# Autodesk Inventor assembly: LCDassembly
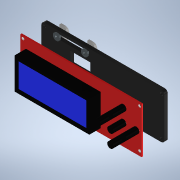
[picture p0: Inventor's stored thumbnail of the model, 180x180]
Saved by Autodesk Inventor 2020.2 (Build 242310000, 310)
## iProperties
Created: 2020-08-24
Part Number: LCDassembly
Document SubType Name: Assembly
Designer: JK
Author: JK
## Documents named in this file (5)
- C:\Users\JK\Documents\Inventor\Anet Upgrade\LCDassembly.iam
- C:\Users\JK\Documents\Inventor\Anet Upgrade\LCDmount.ipt
- C:\Users\JK\Documents\Inventor\Anet Upgrade\LCDScreen.ipt
- C:\Users\JK\Documents\Inventor\Anet Upgrade\M5x12BoltFlatHead.ipt
- C:\Users\JK\Documents\Inventor\Anet Upgrade\T_Slot_Nut_Dropin_3030m5ipt.ipt
## Components (6 placed, 4 different names)
1. LCDmount:1 — Mate:1, Mate:2, Mate:5, Mate:6, Mate:7, Mate:8
2. LCDScreen:1 — Mate:1, Mate:2
3. M5x12BoltFlatHead:1 — Flush:1, Mate:4
4. M5x12BoltFlatHead:2 — Flush:1, Mate:3
5. T_Slot_Nut_Dropin_3030m5ipt:1 — Mate:3, Flush:2, Mate:8, Flush:3
6. T_Slot_Nut_Dropin_3030m5ipt:2 — Mate:4, Flush:2, Mate:5, Mate:6, Mate:7, Flush:3
## Relationships (11: Mate 8, Flush 3)
- Mate:1: LCDmount:1 ↔ LCDScreen:1
- Mate:2: LCDmount:1 ↔ LCDScreen:1
- Flush:1: M5x12BoltFlatHead:1 ↔ M5x12BoltFlatHead:2
- Mate:3: M5x12BoltFlatHead:2 ↔ T_Slot_Nut_Dropin_3030m5ipt:1
- Mate:4: M5x12BoltFlatHead:1 ↔ T_Slot_Nut_Dropin_3030m5ipt:2
- Flush:2: T_Slot_Nut_Dropin_3030m5ipt:1 ↔ T_Slot_Nut_Dropin_3030m5ipt:2
- Mate:5 (-1.5 mm): LCDmount:1 ↔ T_Slot_Nut_Dropin_3030m5ipt:2
- Mate:6: LCDmount:1 ↔ T_Slot_Nut_Dropin_3030m5ipt:2
- Mate:7: LCDmount:1 ↔ T_Slot_Nut_Dropin_3030m5ipt:2
- Mate:8: LCDmount:1 ↔ T_Slot_Nut_Dropin_3030m5ipt:1
- Flush:3: T_Slot_Nut_Dropin_3030m5ipt:1 ↔ T_Slot_Nut_Dropin_3030m5ipt:2
